# Autodesk Inventor assembly: ensamblaje_tension
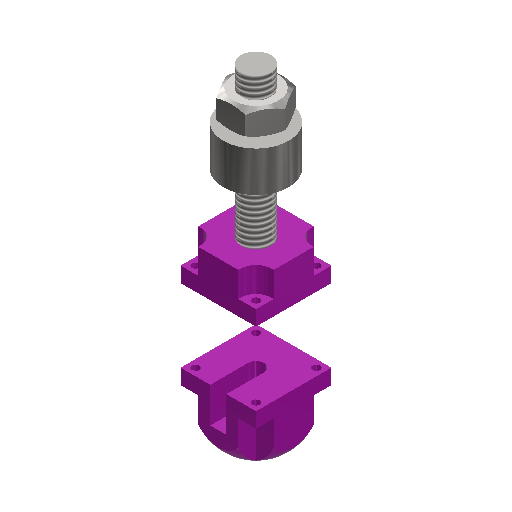
[picture p0: Inventor's stored thumbnail of the model, 512x512]
Saved by Autodesk Inventor 2026.1 (Build 301233000, 233)
## iProperties
Created: 2025-10-01
Part Number: ensamblaje_tension
Document SubType Name: Assembly
Designer: gianm
Author: gianm
## Documents named in this file (5)
- D:\Tesis\Modelo 3D\CAD\Tension\ensamblaje_tension.iam
- D:\Tesis\Modelo 3D\CAD\Tension\sensor_tension.ipt
- D:\Tesis\Modelo 3D\CAD\Tension\Accesorios\ISO 4032 - M6 - ISO.ipt
- D:\Tesis\Modelo 3D\CAD\Tension\sujecion_cable.ipt
- D:\Tesis\Modelo 3D\CAD\Tension\sujecion_cable_2.ipt
## Components (5 placed, 4 different names)
1. sensor_tension:1 — Coincidencia:1, Coincidencia:2, Coincidencia:3, Coincidencia:4
2. ISO 4032 M6:1 — Coincidencia:1
3. ISO 4032 M6:2 — Coincidencia:2
4. sujecion_cable:1 — Coincidencia:3, Nivelación:1
5. sujecion_cable_2:1 — Coincidencia:4, Nivelación:1
## Relationships (5: Mate 4, Flush 1)
- Coincidencia:1 [Mate]: sensor_tension:1 ↔ ISO 4032 M6:1
- Coincidencia:2 [Mate]: sensor_tension:1 ↔ ISO 4032 M6:2
- Coincidencia:3 [Mate]: sensor_tension:1 ↔ sujecion_cable:1
- Coincidencia:4 [Mate]: sensor_tension:1 ↔ sujecion_cable_2:1
- Nivelación:1 [Flush]: sujecion_cable:1 ↔ sujecion_cable_2:1
